# Autodesk Inventor assembly: assrmbly camera
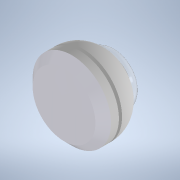
[picture p0: Inventor's stored thumbnail of the model, 180x180]
Saved by Autodesk Inventor 2022.2 (Build 262287000, 287)
## iProperties
Created: 2022-02-22
Part Number: assrmbly camera
Document SubType Name: Assembly
Designer: ONG
Author: ONG
## Documents named in this file (3)
- C:\Users\ONG\Documents\INVENTOR DESIGN\音箱\assrmbly camera.iam
- C:\Users\ONG\Documents\INVENTOR DESIGN\音箱\camera cover.ipt
- C:\Users\ONG\Documents\INVENTOR DESIGN\音箱\camera.ipt
## Components (2 placed, 2 different names)
1. camera cover:1 — Insert:1
2. camera:1 — Insert:1
## Relationships (1: Insert 1)
- Insert:1 (-2 mm): camera cover:1 ↔ camera:1
